# Autodesk Inventor assembly: Stand Assembly
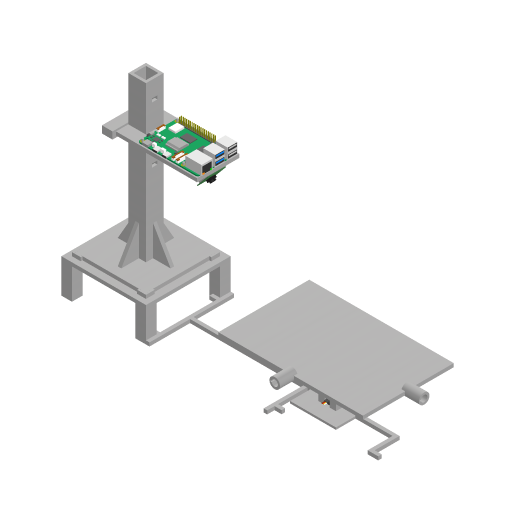
[picture p0: Inventor's stored thumbnail of the model, 512x512]
Saved by Autodesk Inventor 2023.4 (Build 274418000, 418)
## iProperties
Created: 2024-02-27
Part Number: Stand Assembly
Document SubType Name: Assembly
Designer: josep
Author: josep
## iProperties of the stored document SER0044.ipt
Created: 2024-02-13
Part Number: SER0044
Material: Generic
Description: Unknown
Document SubType Name: Modeling
Designer: josep
Authority: Unknown
Density: 1 g/cm^3
Appearance: Default
Company: Unknown
Title: SER0044
Author: Unknown
Sending System: Solid Edge
Preprocessor: ST-DEVELOPER v18.102
## iProperties of the stored document yawmount44.ipt
Created: 2024-03-14
Part Number: yawmount44
Material: Generic
Document SubType Name: Modeling
Designer: josep
Density: 1 g/cm^3
Appearance: Default
Author: josep
Sending System: Autodesk Inventor 2024
## Documents named in this file (15)
- **C:\Users\josep\OneDrive - University of Bath\Documents\University\Year IV\FYP Ideas\Precision Landing\Bench Test\Stand Assembly.iam*LocalDocs*xAaaaaoaaAaaaaaaaAaaaq1f25d*SER0044.ipt
- **C:\Users\josep\OneDrive - University of Bath\Documents\University\Year IV\FYP Ideas\Precision Landing\Bench Test\Stand Assembly.iam*LocalDocs*xAaaaquaaAaaaaaaaAaaaa4ufYg*yawmount44.ipt
- C:\Users\josep\OneDrive - University of Bath\Documents\University\Year IV\FYP Ideas\Precision Landing\Bench Test\Stand Assembly.iam
- C:\Users\josep\OneDrive - University of Bath\Documents\University\Year IV\FYP Ideas\Precision Landing\Bench Test\Fixture.ipt
- C:\Users\josep\OneDrive - University of Bath\Documents\University\Year IV\FYP Ideas\Precision Landing\Bench Test\Platform.ipt
- C:\Users\josep\OneDrive - University of Bath\Documents\University\Year IV\FYP Ideas\Precision Landing\Bench Test\Stand.ipt
- C:\Users\josep\OneDrive - University of Bath\Documents\University\Year IV\FYP Ideas\Precision Landing\Bench Test\GroundCorrected.ipt
- C:\Users\josep\OneDrive - University of Bath\Documents\University\Year IV\FYP Ideas\Precision Landing\Bench Test\Servo Adapter.ipt
- C:\Users\josep\Downloads\raspberry-pi-5-sbc-1.snapshot.2\raspberry-pi-5-sbc-simple\raspberry-pi-5-sbc-simple.ipt
- C:\Users\josep\Downloads\Raspberry Pi  Camera\Raspberry Pi  Camera.ipt
- C:\Users\josep\OneDrive - University of Bath\Documents\University\Year IV\FYP Ideas\Precision Landing\Bench Test\Stand Legs.ipt
- C:\Users\josep\OneDrive - University of Bath\Documents\University\Year IV\FYP Ideas\Precision Landing\Bench Test\yawmount.ipt
- C:\Users\josep\OneDrive - University of Bath\Documents\University\Year IV\FYP Ideas\Precision Landing\Bench Test\Positioning Stencil.ipt
- C:\Users\josep\OneDrive - University of Bath\Documents\University\Year IV\FYP Ideas\Precision Landing\Bench Test\yawmount44.ipt
- C:\Users\josep\Downloads\LIB_SER0044\SER0044\3D\SER0044.stp
## Components (12 placed, 12 different names)
1. Fixture:1 — Mate:4, Mate:5, Mate:6
2. Platform:1 — Mate:1, Mate:2, Mate:3, Mate:5, Mate:6, Rotational:2, Mate:11, Rotational:3, Mate:12, Mate:13
3. Stand:1 — Mate:1, Mate:2, Mate:3, Mate:4, Mate:14, Flush:3, Flush:4
4. GroundCorrected:1 — Rotational:1, Mate:15, Flush:2
5. Servo Adapter:1 — Rotational:1, Insert:1
6. raspberry-pi-5-sbc-simple:1 — Mate:12, Mate:13
7. Raspberry Pi  Camera:1 — Rotational:2, Mate:11, Rotational:3
8. Stand Legs:1 — Mate:14, Mate:15, Flush:2, Flush:3, Flush:4, Mate:16, Mate:17, Mate:23, Mate:25
9. yawmount:1 — Mate:18
10. yawmount44:1 — Mate:19, Mate:21, Mate:22, Angle:1
11. SER0044:1 — Mate:20, Mate:21, Mate:22, Insert:1
12. Positioning Stencil:1 — Mate:23, Mate:24, Mate:25
## Relationships (29: Mate 21, RevoluteJoint 3, Flush 3, Insert 1, Angle 1)
- Mate:1: Platform:1 ↔ Stand:1
- Mate:2: Platform:1 ↔ Stand:1
- Mate:3: Platform:1 ↔ Stand:1
- Mate:4: Fixture:1 ↔ Stand:1
- Mate:5: Fixture:1 ↔ Platform:1
- Mate:6: Fixture:1 ↔ Platform:1
- Rotational:1 [RevoluteJoint]: GroundCorrected:1 ↔ Servo Adapter:1
- Rotational:2 [RevoluteJoint]: Platform:1 ↔ Raspberry Pi  Camera:1
- Mate:11: Platform:1 ↔ Raspberry Pi  Camera:1
- Rotational:3 [RevoluteJoint]: Platform:1 ↔ Raspberry Pi  Camera:1
- Mate:12: Platform:1 ↔ raspberry-pi-5-sbc-simple:1
- Mate:13: Platform:1 ↔ raspberry-pi-5-sbc-simple:1
- Mate:14: Stand:1 ↔ Stand Legs:1
- Mate:15 (107.107 mm): GroundCorrected:1 ↔ Stand Legs:1
- Flush:2 (4.5 mm): GroundCorrected:1 ↔ Stand Legs:1
- Flush:3 (10 mm): Stand:1 ↔ Stand Legs:1
- Flush:4 (10 mm): Stand:1 ↔ Stand Legs:1
- Mate:16: Stand Legs:1
- Mate:17: Stand Legs:1
- Mate:18: yawmount:1
- Mate:19: yawmount44:1
- Mate:20: SER0044:1
- Mate:21: yawmount44:1 ↔ SER0044:1
- Mate:22: yawmount44:1 ↔ SER0044:1
- Insert:1: Servo Adapter:1 ↔ SER0044:1
- Angle:1 (0 deg): yawmount44:1
- Mate:23: Stand Legs:1 ↔ Positioning Stencil:1
- Mate:24: Positioning Stencil:1
- Mate:25: Stand Legs:1 ↔ Positioning Stencil:1
